# Autodesk Inventor assembly: roll_support_right
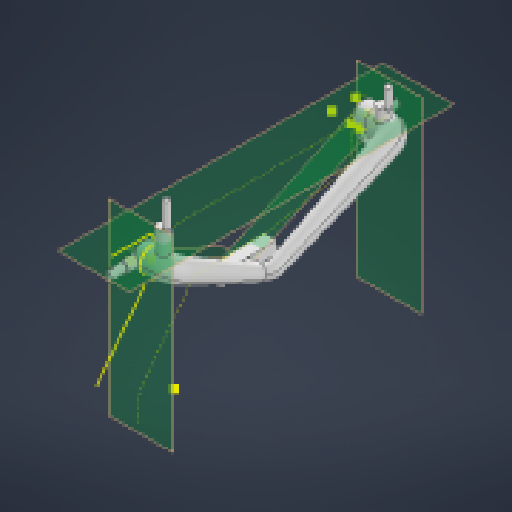
[picture p0: Inventor's stored thumbnail of the model, 512x512]
Saved by Autodesk Inventor 2026.1 (Build 301233020, 233B)
## iProperties
Created: 2025-11-28
Part Number: roll_support_right
Document SubType Name: Assembly
Designer: jaewook
Author: jaewook
## Documents named in this file (3)
- C:\Users\kjh19\Documents\Inventor\project\final\roll_support_right.iam
- C:\Users\kjh19\Documents\Inventor\project\proto2\example\roll_behind_1.ipt
- C:\Users\kjh19\Documents\Inventor\project\proto2\example\base_behind.ipt
## Components (2 placed, 2 different names)
1. roll_behind_1:2 — 메이트:1
2. base_behind:1 — 메이트:1
## Relationships (1: Mate 1)
- 메이트:1 [Mate]: roll_behind_1:2 ↔ base_behind:1
